# Autodesk Inventor assembly: Zinc Alloy Pillow Block Flange Bearing KFL08 ID-8mm
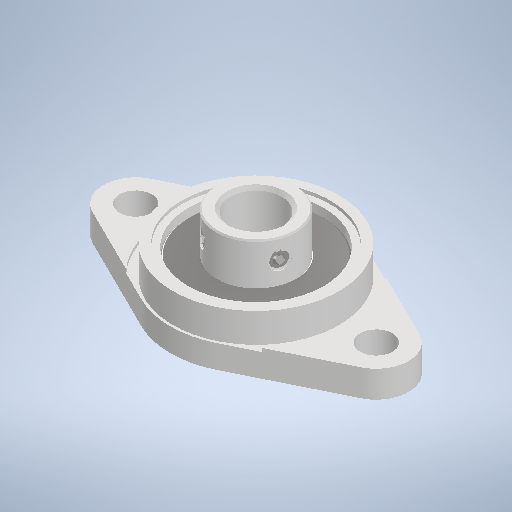
[picture p0: Inventor's stored thumbnail of the model, 512x512]
Saved by Autodesk Inventor 2025.2 (Build 292293000, 293)
## iProperties
Created: 2021-04-20
Part Number: Zinc Alloy Pillow Block Flange Bearing KFL08 ID-8mm
Document SubType Name: Assembly
Designer: Johnson Ebenezer R
Author: Johnson Ebenezer R
## Documents named in this file (6)
- C:\Users\Simon\OneDrive\Documents\Inventor\Skripsie2025\PartsFolder\Pillow Block Bearing 1\Zinc Alloy Pillow Block Flange Bearing KFL08 ID-8mm.iam
- C:\Users\Simon\OneDrive\Documents\Inventor\Skripsie2025\PartsFolder\Pillow Block Bearing 1\Flange.ipt
- C:\Users\Simon\OneDrive\Documents\Inventor\Skripsie2025\PartsFolder\Pillow Block Bearing 1\Bearing 61801-2Z GB_T 276-94.ipt
- C:\Users\Simon\OneDrive\Documents\Inventor\Skripsie2025\PartsFolder\Pillow Block Bearing 1\DIN 988 - 13 x 19 x 1.ipt
- C:\Users\Simon\OneDrive\Documents\Inventor\Skripsie2025\PartsFolder\Pillow Block Bearing 1\Collar 8x12.35x11.35.ipt
- C:\Users\Simon\OneDrive\Documents\Inventor\Skripsie2025\PartsFolder\Pillow Block Bearing 1\IS_ 6094 - M3 x 2FP.ipt
## Components (8 placed, 5 different names)
1. Flange:1 — Mate:1, Flush:1, Mate:7, Mate:8, Mate:9
2. Rolling bearing GB/T 276-1994 Type 60000-2Z 61801-2Z:1 — Mate:1, Flush:1, Mate:2, Mate:3, Mate:4, Mate:5, Flush:2, Mate:6
3. DIN 988 13 x 19 x 1:2 — Mate:2, Mate:5
4. DIN 988 13 x 19 x 1:1 — Mate:3, Mate:4
5. Collar 8x12.35x11.35:1 — Flush:2, Mate:6, Mate:10, Mate:11
6. IS 6094 FP M3 x 2:1 — Mate:10
7. IS 6094 FP M3 x 2:2 — Mate:11
8. IS 6094 FP M3 x 2:3
## Component patterns: (2 elements, first: IS 6094 FP M3 x 2:2)
## Relationships (13: Mate 11, Flush 2)
- Mate:1: Flange:1 ↔ Rolling bearing GB/T 276-1994 Type 60000-2Z 61801-2Z:1
- Flush:1 (1.125 mm): Flange:1 ↔ Rolling bearing GB/T 276-1994 Type 60000-2Z 61801-2Z:1
- Mate:2: Rolling bearing GB/T 276-1994 Type 60000-2Z 61801-2Z:1 ↔ DIN 988 13 x 19 x 1:2
- Mate:3: Rolling bearing GB/T 276-1994 Type 60000-2Z 61801-2Z:1 ↔ DIN 988 13 x 19 x 1:1
- Mate:4: Rolling bearing GB/T 276-1994 Type 60000-2Z 61801-2Z:1 ↔ DIN 988 13 x 19 x 1:1
- Mate:5: Rolling bearing GB/T 276-1994 Type 60000-2Z 61801-2Z:1 ↔ DIN 988 13 x 19 x 1:2
- Flush:2: Rolling bearing GB/T 276-1994 Type 60000-2Z 61801-2Z:1 ↔ Collar 8x12.35x11.35:1
- Mate:6: Rolling bearing GB/T 276-1994 Type 60000-2Z 61801-2Z:1 ↔ Collar 8x12.35x11.35:1
- Mate:7: Flange:1
- Mate:8: Flange:1
- Mate:9: Flange:1
- Mate:10: Collar 8x12.35x11.35:1 ↔ IS 6094 FP M3 x 2:1
- Mate:11: Collar 8x12.35x11.35:1 ↔ IS 6094 FP M3 x 2:2
